# Autodesk Inventor assembly: tr2
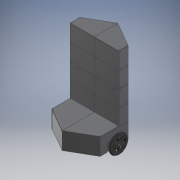
[picture p0: Inventor's stored thumbnail of the model, 180x180]
Saved by Autodesk Inventor 2017 (Build 210142000, 142)
## iProperties
Created: 2018-10-17
Part Number: tr2
Document SubType Name: Assembly
Designer: Administrator
Author: Administrator
## Documents named in this file (3)
- C:\Users\Dell\Documents\GitHub\tr2\TR2.iam
- C:\Users\Dell\Documents\GitHub\tr2\Base\Base.iam
- C:\Users\Dell\Documents\GitHub\tr2\Body\Body.iam
## Components (2 placed, 2 different names)
1. Base:1 [sub-assembly] — Mate:2, Mate:3, Mate:4, Mate:5, Mate:6, Mate:8, Mate:9
2. Body:1 [sub-assembly] — Mate:6, Mate:8, Mate:9
## Relationships (7: Mate 7)
- Mate:2 (40 mm): Base:1
- Mate:3: Base:1
- Mate:4: Base:1
- Mate:5: Base:1
- Mate:6: Base:1 ↔ Body:1
- Mate:8: Base:1 ↔ Body:1
- Mate:9: Base:1 ↔ Body:1
